# Autodesk Inventor assembly: HeadEarConnection
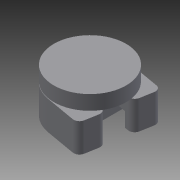
[picture p0: Inventor's stored thumbnail of the model, 180x180]
Saved by Autodesk Inventor 2014 SP1 (Build 180222100, 222)
## iProperties
Created: 2013-10-30
Part Number: HeadEarConnection
Document SubType Name: Assembly
Designer: david
Author: david
## Documents named in this file (3)
- C:\Users\asus\Documents\Autodesk\Projects\SheepWarrior\HeadEarConnection.iam
- C:\Users\asus\Documents\Autodesk\Projects\SheepWarrior\EarConnector.ipt
- C:\Users\asus\Documents\Autodesk\Projects\SheepWarrior\HeadConnector.ipt
## Components (2 placed, 2 different names)
1. EarConnector:1 — Mate:3, Mate:4
2. HeadConnector:1 — Mate:3, Mate:4
## Relationships (2: Mate 2)
- Mate:3: EarConnector:1 ↔ HeadConnector:1
- Mate:4: EarConnector:1 ↔ HeadConnector:1
